# Autodesk Inventor assembly: ___Verkettung
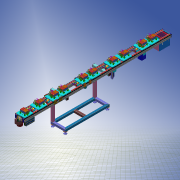
[picture p0: Inventor's stored thumbnail of the model, 180x180]
Saved by Autodesk Inventor 2019 (Build 230136000, 136)
## iProperties
Created: 2023-11-17
Part Number: ___Verkettung
Material: Generisch
Document SubType Name: Assembly
Designer: RP
Source: Unknown
Title: Gurtband WT-240
Author: RP
Revision Number: ANY
## Documents named in this file (10)
- C:\Users\RP\Desktop\__Projekt_Userless_Box\___Projekt_Useless_Box.iam
- C:\Users\RP\Desktop\__Projekt_Userless_Box\_Verkettung\_VK_Hub-Station.iam
- C:\Users\RP\Desktop\__Projekt_Userless_Box\_Verkettung\_VK_Indexier-Station.iam
- C:\Users\RP\Desktop\__Projekt_Userless_Box\_Verkettung\_VK_Hub-Dreh-Station.iam
- C:\Users\RP\Desktop\__Projekt_Userless_Box\_Verkettung\__VK_Stopper.iam
- C:\Users\RP\Desktop\__Projekt_Userless_Box\_Verkettung\_VK_Seitenzentrier-Station.iam
- C:\Users\RP\Desktop\__Projekt_Userless_Box\_Verkettung\__VK_Transferband.iam
- C:\Users\RP\Desktop\__Projekt_Userless_Box\_Verkettung\__VK_Gestell.iam
- C:\Users\RP\Desktop\__Projekt_Userless_Box\_Verkettung\__VK_WT_beladen.iam
- C:\Users\RP\Desktop\__Projekt_Userless_Box\_Verkettung\__VK_Sensor_Palette_1_0.ipt
## Components (20 placed, 9 different names)
1. __VK_Transferband:1 [sub-assembly] — Passend:107, Passend:108, Fluchtend:96, Fluchtend:97, Passend:109, Passend:110, Fluchtend:98, Passend:112, Fluchtend:99, Passend:113, Fluchtend:100, Fluchtend:101, Passend:114
2. __VK_Stopper:7 [sub-assembly] — Fluchtend:86, Fluchtend:91, Passend:105, Passend:111
3. __VK_Sensor_Palette_1_0:1 — Passend:109, Passend:110, Passend:111
4. __VK_WT_beladen:1 [sub-assembly] — Fluchtend:79, Passend:81, Passend:105, Fluchtend:95, Fluchtend:97, Fluchtend:102
5. _VK_Seitenzentrier-Station:1 [sub-assembly] — Fluchtend:87, Fluchtend:88, Passend:97, Passend:98
6. __VK_WT_beladen:2 [sub-assembly] — Fluchtend:89, Passend:91, Passend:97, Fluchtend:94, Fluchtend:95
7. __VK_WT_beladen:3 [sub-assembly] — Fluchtend:9, Passend:92, Passend:98
8. _VK_Indexier-Station:1 [sub-assembly] — Fluchtend:85, Passend:99, Passend:100
9. __VK_WT_beladen:4 [sub-assembly] — Fluchtend:81, Passend:96, Passend:99, Fluchtend:93, Fluchtend:94
10. __VK_WT_beladen:5 [sub-assembly] — Fluchtend:23, Passend:93, Passend:100
11. _VK_Hub-Station:1 [sub-assembly] — Fluchtend:84, Passend:101, Passend:102
12. __VK_WT_beladen:6 [sub-assembly] — Fluchtend:67, Passend:95, Passend:101, Fluchtend:92, Fluchtend:93
13. __VK_WT_beladen:7 [sub-assembly] — Fluchtend:76, Passend:94, Passend:102
14. _VK_Hub-Dreh-Station:1 [sub-assembly] — Fluchtend:83, Passend:103, Passend:104
15. __VK_WT_beladen:8 [sub-assembly] — Passend:82, Fluchtend:82, Passend:103, Fluchtend:92
16. __VK_WT_beladen:9 [sub-assembly] — Fluchtend:80, Passend:80, Passend:104
17. __VK_Gestell:2 [sub-assembly] — Passend:108, Fluchtend:96
18. __VK_Transferband:2 [sub-assembly] — Fluchtend:98, Passend:112, Fluchtend:99
19. __VK_Transferband:3 [sub-assembly] — Passend:113, Fluchtend:100, Fluchtend:101
20. __VK_WT_beladen:10 [sub-assembly] — Passend:114, Fluchtend:102
## Relationships (61: Flush 32, Mate 29)
- [Mate]: __VK_Transferband:1
- [Mate]: __VK_Transferband:1
- [Flush]: __VK_Transferband:1
- [Mate]: __VK_Transferband:1
- Fluchtend:9 [Flush]: __VK_WT_beladen:3
- Fluchtend:23 [Flush]: __VK_WT_beladen:5
- Fluchtend:81 [Flush]: __VK_WT_beladen:4
- Fluchtend:67 [Flush]: __VK_WT_beladen:6
- [Flush]: _VK_Hub-Station:1
- [Flush]: _VK_Indexier-Station:1
- [Flush]: _VK_Hub-Dreh-Station:1
- Fluchtend:76 [Flush]: __VK_WT_beladen:7
- Fluchtend:79 [Flush]: __VK_WT_beladen:1
- Fluchtend:80 [Flush]: __VK_WT_beladen:9
- Passend:80 [Mate]: __VK_WT_beladen:9
- Passend:81 [Mate]: __VK_WT_beladen:1
- Passend:82 [Mate]: __VK_WT_beladen:8
- Fluchtend:82 [Flush]: __VK_WT_beladen:8
- Fluchtend:83 [Flush]: _VK_Hub-Dreh-Station:1
- Fluchtend:84 [Flush]: _VK_Hub-Station:1
- Fluchtend:85 [Flush]: _VK_Indexier-Station:1
- Fluchtend:86 [Flush]: __VK_Stopper:7
- Fluchtend:87 [Flush]: _VK_Seitenzentrier-Station:1
- Fluchtend:88 [Flush]: _VK_Seitenzentrier-Station:1
- Fluchtend:89 [Flush]: __VK_WT_beladen:2
- Passend:91 [Mate]: __VK_WT_beladen:2
- [Flush]: __VK_Transferband:1
- Passend:92 [Mate]: __VK_WT_beladen:3
- Passend:93 [Mate]: __VK_WT_beladen:5
- Passend:94 [Mate]: __VK_WT_beladen:7
- Passend:95 [Mate]: __VK_WT_beladen:6
- Passend:96 [Mate]: __VK_WT_beladen:4
- Passend:97 [Mate]: _VK_Seitenzentrier-Station:1 ↔ __VK_WT_beladen:2
- Passend:98 [Mate]: _VK_Seitenzentrier-Station:1 ↔ __VK_WT_beladen:3
- Passend:99 [Mate]: _VK_Indexier-Station:1 ↔ __VK_WT_beladen:4
- Passend:100 [Mate]: _VK_Indexier-Station:1 ↔ __VK_WT_beladen:5
- Passend:101 [Mate]: _VK_Hub-Station:1 ↔ __VK_WT_beladen:6
- Passend:102 [Mate]: _VK_Hub-Station:1 ↔ __VK_WT_beladen:7
- Passend:103 [Mate]: _VK_Hub-Dreh-Station:1 ↔ __VK_WT_beladen:8
- Passend:104 [Mate]: _VK_Hub-Dreh-Station:1 ↔ __VK_WT_beladen:9
- Fluchtend:91 [Flush]: __VK_Stopper:7
- Passend:105 [Mate]: __VK_Stopper:7 ↔ __VK_WT_beladen:1
- Passend:107 [Mate]: __VK_Transferband:1
- Fluchtend:92 [Flush] (800 mm): __VK_WT_beladen:6 ↔ __VK_WT_beladen:8
- Fluchtend:93 [Flush] (800 mm): __VK_WT_beladen:4 ↔ __VK_WT_beladen:6
- Fluchtend:94 [Flush] (800 mm): __VK_WT_beladen:2 ↔ __VK_WT_beladen:4
- Fluchtend:95 [Flush] (400 mm): __VK_WT_beladen:1 ↔ __VK_WT_beladen:2
- Passend:108 [Mate]: __VK_Transferband:1 ↔ __VK_Gestell:2
- Fluchtend:96 [Flush]: __VK_Transferband:1 ↔ __VK_Gestell:2
- Fluchtend:97 [Flush] (400 mm): __VK_Transferband:1 ↔ __VK_WT_beladen:1
- Passend:109 [Mate]: __VK_Transferband:1 ↔ __VK_Sensor_Palette_1_0:1
- Passend:110 [Mate]: __VK_Transferband:1 ↔ __VK_Sensor_Palette_1_0:1
- Passend:111 [Mate]: __VK_Stopper:7 ↔ __VK_Sensor_Palette_1_0:1
- Fluchtend:98 [Flush]: __VK_Transferband:1 ↔ __VK_Transferband:2
- Passend:112 [Mate]: __VK_Transferband:1 ↔ __VK_Transferband:2
- Fluchtend:99 [Flush]: __VK_Transferband:1 ↔ __VK_Transferband:2
- Passend:113 [Mate]: __VK_Transferband:1 ↔ __VK_Transferband:3
- Fluchtend:100 [Flush]: __VK_Transferband:1 ↔ __VK_Transferband:3
- Fluchtend:101 [Flush]: __VK_Transferband:1 ↔ __VK_Transferband:3
- Passend:114 [Mate]: __VK_Transferband:1 ↔ __VK_WT_beladen:10
- Fluchtend:102 [Flush]: __VK_WT_beladen:1 ↔ __VK_WT_beladen:10
